# Autodesk Inventor assembly: Noise_ASM
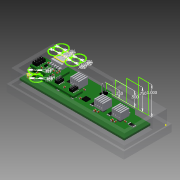
[picture p0: Inventor's stored thumbnail of the model, 180x180]
Saved by Autodesk Inventor 2014 (Build 180170000, 170)
## iProperties
Created: 2015-11-05
Part Number: Noise_ASM
Document SubType Name: Assembly
Designer: Owner
Author: Owner
## Documents named in this file (23)
- C:\Users\Owner\Documents\APC\FrontEnd\IAM\Common\NoiseSource\Noise_ASM.iam
- C:\Users\Owner\Documents\APC\FrontEnd\IAM\Common\NoiseSource\MezzanineBoard.ipt
- C:\Users\Owner\Documents\APC\FrontEnd\IAM\Common\NoiseSource\NoiseBoard.ipt
- C:\Users\Owner\Documents\APC\FrontEnd\IAM\Common\NoiseSource\Header_127.ipt
- C:\Users\Owner\Documents\APC\FrontEnd\IAM\Common\FirstStageAmp.ipt
- C:\Users\Owner\Documents\APC\FrontEnd\IAM\Common\RFSwitch.ipt
- C:\Users\Owner\Documents\APC\FrontEnd\IAM\Common\UMCC.ipt
- C:\Users\Owner\Documents\APC\FrontEnd\IAM\Common\2mm4PosHeader.ipt
- C:\Users\Owner\Documents\APC\FrontEnd\IAM\Common\2mm2Row8PosFemale.ipt
- C:\Users\Owner\Documents\APC\FrontEnd\IAM\Common\Block.ipt
- C:\Users\Owner\Documents\APC\FrontEnd\IAM\Common\2020Resistor.ipt
- C:\Users\Owner\Documents\APC\FrontEnd\IAM\Common\0806Cap.ipt
- C:\Users\Owner\Documents\APC\FrontEnd\IAM\Common\0603Inductor.ipt
- C:\Users\Owner\Documents\APC\FrontEnd\IAM\Common\0603Cap.ipt
- C:\Users\Owner\Documents\APC\FrontEnd\IAM\Common\SmallHeatsink.ipt
- C:\Users\Owner\Documents\APC\FrontEnd\IAM\Common\127mm2Row8PosFemale.ipt
- C:\Users\Owner\Documents\APC\FrontEnd\IAM\Common\2mmWireBoardConn.ipt
- C:\Users\Owner\Documents\APC\FrontEnd\IAM\Common\2mmWireBoardConn_plug.ipt
- C:\Users\Owner\Documents\APC\FrontEnd\IAM\Common\0603Resistor.ipt
- C:\Users\Owner\Documents\APC\FrontEnd\IAM\Common\DualNotGate.ipt
- C:\Users\Owner\Documents\APC\FrontEnd\IAM\Common\UMCC_Plug.ipt
- C:\Users\Owner\Documents\APC\FrontEnd\IAM\Common\2PinHeader.ipt
- C:\Users\Owner\Documents\APC\FrontEnd\IAM\Common\NoiseSourceWell.ipt
## Components (71 placed, 22 different names)
1. MezzanineBoard:1 — Mate:5, Mate:14, Mate:15, Mate:16, Mate:53, Mate:54, Mate:55, Mate:56, Mate:57, Mate:58, Mate:66, Mate:67, Angle:1, Mate:68, Mate:69, Mate:70, Mate:71, Mate:72, Mate:73, Flush:92, Flush:93, Flush:94, Flush:95, Flush:96, Flush:97, Flush:98, Flush:99, Flush:100, Flush:101, Flush:102, Flush:103, Mate:74, Mate:75, Mate:76, Flush:104, Flush:105, Flush:106, Flush:107, Flush:108, Flush:109, Mate:77, Mate:78, Mate:79, Mate:80, Flush:110, Flush:111, Flush:112, Flush:113, Flush:114, Flush:115, Flush:116, Flush:117
2. NoiseBoard:1 — Mate:1, Mate:2, Flush:1, Flush:2, Flush:3, Flush:4, Mate:6, Mate:7, Mate:8, Mate:9, Mate:10, Mate:11, Mate:12, Flush:11, Flush:12, Flush:13, Flush:14, Flush:15, Flush:16, Flush:17, Flush:18, Flush:19, Flush:20, Flush:21, Flush:22, Flush:23, Flush:24, Mate:13, Tangent:1, Tangent:2, Flush:25, Mate:17, Mate:18, Mate:19, Mate:20, Mate:21, Flush:26, Flush:27, Flush:28, Flush:29, Flush:30, Flush:31, Flush:32, Flush:33, Flush:34, Flush:35, Mate:22, Mate:23, Mate:24, Mate:25, Mate:26, Mate:27, Flush:36, Flush:37, Flush:38, Flush:39, Flush:40, Flush:41, Flush:42, Flush:43, Flush:44, Flush:45, Flush:46, Flush:47, Mate:28, Mate:29, Mate:30, Mate:31, Mate:32, Mate:33, Flush:48, Flush:49, Flush:50, Flush:51, Flush:52, Flush:53, Flush:54, Flush:55, Flush:56, Flush:57, Flush:58, Flush:59, Mate:34, Mate:35, Mate:36, Mate:37, Mate:38, Mate:39, Mate:40, Mate:41, Mate:42, Mate:43, Mate:44, Flush:60, Flush:61, Flush:62, Flush:63, Flush:64, Flush:65, Flush:66, Flush:67, Flush:68, Flush:69, Flush:70, Flush:71, Flush:72, Flush:73, Flush:74, Flush:75, Flush:76, Flush:77, Flush:78, Flush:79, Flush:80, Flush:81, Mate:45, Mate:46, Mate:47, Mate:48, Mate:49, Flush:82, Flush:83, Flush:84, Flush:85, Flush:86, Flush:87, Flush:88, Flush:89, Flush:90, Flush:91, Mate:83, Flush:118, Flush:119
3. Header_127:1 — Mate:1, Flush:2, Flush:4, Mate:5, Mate:59, Mate:60
4. Header_127:2 — Mate:2, Flush:1, Flush:3
5. UMCC:1 — Mate:12, Flush:11, Flush:12, Mate:81, Mate:82
6. 2mm4PosHeader:1 — Mate:13, Tangent:1, Tangent:2
7. 2mm2Row8PosFemale:1 — Mate:14, Mate:15, Mate:16
8. Block:1 — Flush:25
9. SmallHeatsink:1 — Mate:50
10. SmallHeatsink:2 — Mate:51
11. SmallHeatsink:3 — Mate:52
12. 127mm2Row8PosFemale:1 — Mate:53, Mate:56, Mate:58
13. 127mm2Row8PosFemale:2 — Mate:54, Mate:55, Mate:57, Mate:59, Mate:60
14. 2mmWireBoardConn:1 — Mate:63, Mate:64, Mate:65, Mate:66, Mate:67, Angle:1
15. 2mmWireBoardConn_plug:1 — Mate:63, Mate:64, Mate:65, Mate:84, Flush:120, Flush:121
16. 0603Resistor:1 — Mate:68, Flush:92, Flush:98
17. 0603Resistor:2 — Mate:69, Flush:93, Flush:100
18. 0603Cap:17 — Mate:70, Flush:95, Flush:99
19. 0603Cap:18 — Mate:71, Flush:96, Flush:101
20. 0603Cap:19 — Mate:73, Flush:97, Flush:103
21. 0603Cap:20 — Mate:72, Flush:94, Flush:102
22. DualNotGate:1 — Mate:75, Flush:105, Flush:107
23. DualNotGate:2 — Mate:76, Flush:104, Flush:109
24. DualNotGate:3 — Mate:74, Flush:106, Flush:108
25. 0603Cap:21 — Mate:77, Flush:116, Flush:117
26. 0603Cap:22 — Mate:78, Flush:114, Flush:115
27. 0603Cap:23 — Mate:79, Flush:112, Flush:113
28. 0603Cap:24 — Mate:80, Flush:110, Flush:111
29. UMCC_Plug:1 — Mate:81, Mate:82
30. 2PinHeader:1 — Mate:83, Flush:118, Flush:119
31. 2mmWireBoardConn_plug:2 — Mate:84, Flush:120, Flush:121
32. NoiseSourceWell:1
33. FirstStageAmp:3 — Mate:8, Flush:22, Flush:24, Mate:52
34. FirstStageAmp:2 — Mate:7, Flush:19, Flush:20, Mate:51
35. FirstStageAmp:1 — Mate:6, Flush:21, Flush:23, Mate:50
36. 2020Resistor:2 — Mate:18, Flush:30, Flush:32
37. 2020Resistor:3 — Mate:19, Flush:34, Flush:35
38. 2020Resistor:4 — Mate:20, Flush:28, Flush:29
39. 0806Cap:1 — Mate:22, Flush:36, Flush:37
40. 0806Cap:2 — Mate:23, Flush:46, Flush:47
41. 0806Cap:3 — Mate:24, Flush:40, Flush:41
42. 0806Cap:4 — Mate:25, Flush:44, Flush:45
43. 0806Cap:5 — Mate:27, Flush:42, Flush:43
44. 0806Cap:6 — Mate:26, Flush:38, Flush:39
45. 0603Inductor:1 — Mate:33, Flush:48, Flush:49
46. 0603Inductor:2 — Mate:32, Flush:50, Flush:51
47. 0603Inductor:3 — Mate:31, Flush:52, Flush:54
48. 0603Inductor:4 — Mate:30, Flush:53, Flush:55
49. 0603Inductor:5 — Mate:29, Flush:56, Flush:58
50. 0603Inductor:6 — Mate:28, Flush:57, Flush:59
51. 0603Cap:1 — Mate:40, Flush:62, Flush:65
52. 0603Cap:2 — Mate:38, Flush:67, Flush:69
53. 0603Cap:3 — Mate:39, Flush:70, Flush:73
54. 0603Cap:4 — Mate:37, Flush:74, Flush:76
55. 0603Cap:5 — Mate:35, Flush:75, Flush:77
56. 0603Cap:6 — Mate:36, Flush:80, Flush:81
57. 0603Cap:7 — Mate:34, Flush:78, Flush:79
58. 0603Cap:8 — Mate:41, Flush:61, Flush:64
59. 0603Cap:9 — Mate:42, Flush:66, Flush:68
60. 0603Cap:10 — Mate:43, Flush:71, Flush:72
61. 0603Cap:11 — Mate:44, Flush:60, Flush:63
62. RFSwitch:2 — Mate:10, Flush:15, Flush:16
63. RFSwitch:1 — Mate:11, Flush:13, Flush:14
64. 0603Cap:12 — Mate:45, Flush:85, Flush:87
65. 0603Cap:15 — Mate:48, Flush:84, Flush:86
66. 0603Cap:13 — Mate:46, Flush:88, Flush:91
67. 0603Cap:14 — Mate:47, Flush:89, Flush:90
68. RFSwitch:3 — Mate:9, Flush:17, Flush:18
69. 2020Resistor:1 — Mate:17, Flush:26, Flush:27
70. 2020Resistor:5 — Mate:21, Flush:31, Flush:33
71. 0603Cap:16 — Mate:49, Flush:82, Flush:83
## Relationships (198: Flush 115, Mate 80, Tangent 2, Angle 1)
- Mate:1: NoiseBoard:1 ↔ Header_127:1
- Mate:2: NoiseBoard:1 ↔ Header_127:2
- Flush:1 (24.5364 mm): NoiseBoard:1 ↔ Header_127:2
- Flush:2 (37.3126 mm): NoiseBoard:1 ↔ Header_127:1
- Flush:3 (6.7564 mm): NoiseBoard:1 ↔ Header_127:2
- Flush:4 (6.8072 mm): NoiseBoard:1 ↔ Header_127:1
- Mate:5: MezzanineBoard:1 ↔ Header_127:1
- Mate:6: NoiseBoard:1 ↔ FirstStageAmp:1
- Mate:7: NoiseBoard:1 ↔ FirstStageAmp:2
- Mate:8: NoiseBoard:1 ↔ FirstStageAmp:3
- Mate:9: NoiseBoard:1 ↔ RFSwitch:3
- Mate:10: NoiseBoard:1 ↔ RFSwitch:2
- Mate:11: NoiseBoard:1 ↔ RFSwitch:1
- Mate:12: NoiseBoard:1 ↔ UMCC:1
- Flush:11 (4.5212 mm): NoiseBoard:1 ↔ UMCC:1
- Flush:12 (2.3368 mm): NoiseBoard:1 ↔ UMCC:1
- Flush:13 (10.5664 mm): NoiseBoard:1 ↔ RFSwitch:1
- Flush:14 (9.0424 mm): NoiseBoard:1 ↔ RFSwitch:1
- Flush:15 (10.5664 mm): NoiseBoard:1 ↔ RFSwitch:2
- Flush:16 (15.1384 mm): NoiseBoard:1 ↔ RFSwitch:2
- Flush:17 (11.0744 mm): NoiseBoard:1 ↔ RFSwitch:3
- Flush:18 (44.6024 mm): NoiseBoard:1 ↔ RFSwitch:3
- Flush:19 (17.1958 mm): NoiseBoard:1 ↔ FirstStageAmp:2
- Flush:20 (33.0962 mm): NoiseBoard:1 ↔ FirstStageAmp:2
- Flush:21 (10.7442 mm): NoiseBoard:1 ↔ FirstStageAmp:1
- Flush:22 (10.7442 mm): NoiseBoard:1 ↔ FirstStageAmp:3
- Flush:23 (61.2648 mm): NoiseBoard:1 ↔ FirstStageAmp:1
- Flush:24 (76.5302 mm): NoiseBoard:1 ↔ FirstStageAmp:3
- Mate:13: NoiseBoard:1 ↔ 2mm4PosHeader:1
- Mate:14: MezzanineBoard:1 ↔ 2mm2Row8PosFemale:1
- Mate:15 (-1.4224 mm): MezzanineBoard:1 ↔ 2mm2Row8PosFemale:1
- Mate:16 (-2.3114 mm): MezzanineBoard:1 ↔ 2mm2Row8PosFemale:1
- Tangent:1 (-12.2134 mm): NoiseBoard:1 ↔ 2mm4PosHeader:1
- Tangent:2 (-1.7232 mm): NoiseBoard:1 ↔ 2mm4PosHeader:1
- Flush:25: NoiseBoard:1 ↔ Block:1
- Mate:17: NoiseBoard:1 ↔ 2020Resistor:1
- Mate:18: NoiseBoard:1 ↔ 2020Resistor:2
- Mate:19: NoiseBoard:1 ↔ 2020Resistor:3
- Mate:20: NoiseBoard:1 ↔ 2020Resistor:4
- Mate:21: NoiseBoard:1 ↔ 2020Resistor:5
- Flush:26 (17.3482 mm): NoiseBoard:1 ↔ 2020Resistor:1
- Flush:27 (9.8044 mm): NoiseBoard:1 ↔ 2020Resistor:1
- Flush:28 (16.8402 mm): NoiseBoard:1 ↔ 2020Resistor:4
- Flush:29 (24.2824 mm): NoiseBoard:1 ↔ 2020Resistor:4
- Flush:30 (52.451 mm): NoiseBoard:1 ↔ 2020Resistor:2
- Flush:31 (84.6582 mm): NoiseBoard:1 ↔ 2020Resistor:5
- Flush:32 (10.3886 mm): NoiseBoard:1 ↔ 2020Resistor:2
- Flush:33 (12.2174 mm): NoiseBoard:1 ↔ 2020Resistor:5
- Flush:34 (10.3632 mm): NoiseBoard:1 ↔ 2020Resistor:3
- Flush:35 (67.7164 mm): NoiseBoard:1 ↔ 2020Resistor:3
- Mate:22: NoiseBoard:1 ↔ 0806Cap:1
- Mate:23: NoiseBoard:1 ↔ 0806Cap:2
- Mate:24: NoiseBoard:1 ↔ 0806Cap:3
- Mate:25: NoiseBoard:1 ↔ 0806Cap:4
- Mate:26: NoiseBoard:1 ↔ 0806Cap:6
- Mate:27: NoiseBoard:1 ↔ 0806Cap:5
- Flush:36 (30.861 mm): NoiseBoard:1 ↔ 0806Cap:1
- Flush:37 (13.208 mm): NoiseBoard:1 ↔ 0806Cap:1
- Flush:38 (29.591 mm): NoiseBoard:1 ↔ 0806Cap:6
- Flush:39 (24.511 mm): NoiseBoard:1 ↔ 0806Cap:6
- Flush:40 (6.5024 mm): NoiseBoard:1 ↔ 0806Cap:3
- Flush:41 (59.055 mm): NoiseBoard:1 ↔ 0806Cap:3
- Flush:42 (20.701 mm): NoiseBoard:1 ↔ 0806Cap:5
- Flush:43 (58.0644 mm): NoiseBoard:1 ↔ 0806Cap:5
- Flush:44 (6.731 mm): NoiseBoard:1 ↔ 0806Cap:4
- Flush:45 (74.295 mm): NoiseBoard:1 ↔ 0806Cap:4
- Flush:46 (20.2946 mm): NoiseBoard:1 ↔ 0806Cap:2
- Flush:47 (75.565 mm): NoiseBoard:1 ↔ 0806Cap:2
- Mate:28: NoiseBoard:1 ↔ 0603Inductor:6
- Mate:29: NoiseBoard:1 ↔ 0603Inductor:5
- Mate:30: NoiseBoard:1 ↔ 0603Inductor:4
- Mate:31: NoiseBoard:1 ↔ 0603Inductor:3
- Mate:32: NoiseBoard:1 ↔ 0603Inductor:2
- Mate:33: NoiseBoard:1 ↔ 0603Inductor:1
- Flush:48 (19.3548 mm): NoiseBoard:1 ↔ 0603Inductor:1
- Flush:49 (31.0388 mm): NoiseBoard:1 ↔ 0603Inductor:1
- Flush:50 (22.5298 mm): NoiseBoard:1 ↔ 0603Inductor:2
- Flush:51 (32.2326 mm): NoiseBoard:1 ↔ 0603Inductor:2
- Flush:52 (12.9032 mm): NoiseBoard:1 ↔ 0603Inductor:3
- Flush:53 (12.9032 mm): NoiseBoard:1 ↔ 0603Inductor:4
- Flush:54 (59.2074 mm): NoiseBoard:1 ↔ 0603Inductor:3
- Flush:55 (74.4728 mm): NoiseBoard:1 ↔ 0603Inductor:4
- Flush:56 (16.0782 mm): NoiseBoard:1 ↔ 0603Inductor:5
- Flush:57 (16.0782 mm): NoiseBoard:1 ↔ 0603Inductor:6
- Flush:58 (60.4012 mm): NoiseBoard:1 ↔ 0603Inductor:5
- Flush:59 (75.6666 mm): NoiseBoard:1 ↔ 0603Inductor:6
- Mate:34: NoiseBoard:1 ↔ 0603Cap:7
- Mate:35: NoiseBoard:1 ↔ 0603Cap:5
- Mate:36: NoiseBoard:1 ↔ 0603Cap:6
- Mate:37: NoiseBoard:1 ↔ 0603Cap:4
- Mate:38: NoiseBoard:1 ↔ 0603Cap:2
- Mate:39: NoiseBoard:1 ↔ 0603Cap:3
- Mate:40: NoiseBoard:1 ↔ 0603Cap:1
- Mate:41: NoiseBoard:1 ↔ 0603Cap:8
- Mate:42: NoiseBoard:1 ↔ 0603Cap:9
- Mate:43: NoiseBoard:1 ↔ 0603Cap:10
- Mate:44: NoiseBoard:1 ↔ 0603Cap:11
- Flush:60 (12.827 mm): NoiseBoard:1 ↔ 0603Cap:11
- Flush:61 (12.827 mm): NoiseBoard:1 ↔ 0603Cap:8
- Flush:62 (12.827 mm): NoiseBoard:1 ↔ 0603Cap:1
- Flush:63 (80.8228 mm): NoiseBoard:1 ↔ 0603Cap:11
- Flush:64 (71.1708 mm): NoiseBoard:1 ↔ 0603Cap:8
- Flush:65 (55.9054 mm): NoiseBoard:1 ↔ 0603Cap:1
- Flush:66 (7.6708 mm): NoiseBoard:1 ↔ 0603Cap:9
- Flush:67 (7.6708 mm): NoiseBoard:1 ↔ 0603Cap:2
- Flush:68 (76.8858 mm): NoiseBoard:1 ↔ 0603Cap:9
- Flush:69 (61.5188 mm): NoiseBoard:1 ↔ 0603Cap:2
- Flush:70 (18.1864 mm): NoiseBoard:1 ↔ 0603Cap:3
- Flush:71 (18.1864 mm): NoiseBoard:1 ↔ 0603Cap:10
- Flush:72 (75.7428 mm): NoiseBoard:1 ↔ 0603Cap:10
- Flush:73 (60.4774 mm): NoiseBoard:1 ↔ 0603Cap:3
- Flush:74 (19.304 mm): NoiseBoard:1 ↔ 0603Cap:4
- Flush:75 (19.304 mm): NoiseBoard:1 ↔ 0603Cap:5
- Flush:76 (37.6428 mm): NoiseBoard:1 ↔ 0603Cap:4
- Flush:77 (27.7368 mm): NoiseBoard:1 ↔ 0603Cap:5
- Flush:78 (14.1478 mm): NoiseBoard:1 ↔ 0603Cap:7
- Flush:79 (33.4518 mm): NoiseBoard:1 ↔ 0603Cap:7
- Flush:80 (24.4348 mm): NoiseBoard:1 ↔ 0603Cap:6
- Flush:81 (32.1818 mm): NoiseBoard:1 ↔ 0603Cap:6
- Mate:45: NoiseBoard:1 ↔ 0603Cap:12
- Mate:46: NoiseBoard:1 ↔ 0603Cap:13
- Mate:47: NoiseBoard:1 ↔ 0603Cap:14
- Mate:48: NoiseBoard:1 ↔ 0603Cap:15
- Mate:49: NoiseBoard:1 ↔ 0603Cap:16
- Flush:82 (4.4958 mm): NoiseBoard:1 ↔ 0603Cap:16
- Flush:83 (6.5786 mm): NoiseBoard:1 ↔ 0603Cap:16
- Flush:84 (10.8966 mm): NoiseBoard:1 ↔ 0603Cap:15
- Flush:85 (10.8966 mm): NoiseBoard:1 ↔ 0603Cap:12
- Flush:86 (3.6576 mm): NoiseBoard:1 ↔ 0603Cap:15
- Flush:87 (5.715 mm): NoiseBoard:1 ↔ 0603Cap:12
- Flush:88 (13.2588 mm): NoiseBoard:1 ↔ 0603Cap:13
- Flush:89 (10.1346 mm): NoiseBoard:1 ↔ 0603Cap:14
- Flush:90 (42.799 mm): NoiseBoard:1 ↔ 0603Cap:14
- Flush:91 (19.9898 mm): NoiseBoard:1 ↔ 0603Cap:13
- Mate:50 (2 mm): SmallHeatsink:1 ↔ FirstStageAmp:1
- Mate:51 (2 mm): SmallHeatsink:2 ↔ FirstStageAmp:2
- Mate:52 (2 mm): SmallHeatsink:3 ↔ FirstStageAmp:3
- Mate:53: MezzanineBoard:1 ↔ 127mm2Row8PosFemale:1
- Mate:54: MezzanineBoard:1 ↔ 127mm2Row8PosFemale:2
- Mate:55 (-2.6924 mm): MezzanineBoard:1 ↔ 127mm2Row8PosFemale:2
- Mate:56 (-2.6416 mm): MezzanineBoard:1 ↔ 127mm2Row8PosFemale:1
- Mate:57 (-3.5814 mm): MezzanineBoard:1 ↔ 127mm2Row8PosFemale:2
- Mate:58 (-16.3576 mm): MezzanineBoard:1 ↔ 127mm2Row8PosFemale:1
- Mate:59 (0.075 mm): Header_127:1 ↔ 127mm2Row8PosFemale:2
- Mate:60 (0.075 mm): Header_127:1 ↔ 127mm2Row8PosFemale:2
- Mate:63: 2mmWireBoardConn:1 ↔ 2mmWireBoardConn_plug:1
- Mate:64: 2mmWireBoardConn:1 ↔ 2mmWireBoardConn_plug:1
- Mate:65: 2mmWireBoardConn:1 ↔ 2mmWireBoardConn_plug:1
- Mate:66: MezzanineBoard:1 ↔ 2mmWireBoardConn:1
- Mate:67: MezzanineBoard:1 ↔ 2mmWireBoardConn:1
- Angle:1 (0 deg): MezzanineBoard:1 ↔ 2mmWireBoardConn:1
- Mate:68: MezzanineBoard:1 ↔ 0603Resistor:1
- Mate:69: MezzanineBoard:1 ↔ 0603Resistor:2
- Mate:70: MezzanineBoard:1 ↔ 0603Cap:17
- Mate:71: MezzanineBoard:1 ↔ 0603Cap:18
- Mate:72: MezzanineBoard:1 ↔ 0603Cap:20
- Mate:73: MezzanineBoard:1 ↔ 0603Cap:19
- Flush:92 (7.239 mm): MezzanineBoard:1 ↔ 0603Resistor:1
- Flush:93 (7.239 mm): MezzanineBoard:1 ↔ 0603Resistor:2
- Flush:94 (7.239 mm): MezzanineBoard:1 ↔ 0603Cap:20
- Flush:95 (5.207 mm): MezzanineBoard:1 ↔ 0603Cap:17
- Flush:96 (5.207 mm): MezzanineBoard:1 ↔ 0603Cap:18
- Flush:97 (5.207 mm): MezzanineBoard:1 ↔ 0603Cap:19
- Flush:98 (11.8618 mm): MezzanineBoard:1 ↔ 0603Resistor:1
- Flush:99 (11.8618 mm): MezzanineBoard:1 ↔ 0603Cap:17
- Flush:100 (14.986 mm): MezzanineBoard:1 ↔ 0603Resistor:2
- Flush:101 (14.986 mm): MezzanineBoard:1 ↔ 0603Cap:18
- Flush:102 (18.034 mm): MezzanineBoard:1 ↔ 0603Cap:20
- Flush:103 (18.034 mm): MezzanineBoard:1 ↔ 0603Cap:19
- Mate:74: MezzanineBoard:1 ↔ DualNotGate:3
- Mate:75: MezzanineBoard:1 ↔ DualNotGate:1
- Mate:76: MezzanineBoard:1 ↔ DualNotGate:2
- Flush:104 (3.9608 mm): MezzanineBoard:1 ↔ DualNotGate:2
- Flush:105 (2.2082 mm): MezzanineBoard:1 ↔ DualNotGate:1
- Flush:106 (5.2562 mm): MezzanineBoard:1 ↔ DualNotGate:3
- Flush:107 (11.5284 mm): MezzanineBoard:1 ↔ DualNotGate:1
- Flush:108 (7.2104 mm): MezzanineBoard:1 ↔ DualNotGate:3
- Flush:109 (2.5876 mm): MezzanineBoard:1 ↔ DualNotGate:2
- Mate:77: MezzanineBoard:1 ↔ 0603Cap:21
- Mate:78: MezzanineBoard:1 ↔ 0603Cap:22
- Mate:79: MezzanineBoard:1 ↔ 0603Cap:23
- Mate:80: MezzanineBoard:1 ↔ 0603Cap:24
- Flush:110 (6.731 mm): MezzanineBoard:1 ↔ 0603Cap:24
- Flush:111 (2.4638 mm): MezzanineBoard:1 ↔ 0603Cap:24
- Flush:112 (7.2898 mm): MezzanineBoard:1 ↔ 0603Cap:23
- Flush:113 (2.159 mm): MezzanineBoard:1 ↔ 0603Cap:23
- Flush:114 (17.7038 mm): MezzanineBoard:1 ↔ 0603Cap:22
- Flush:115 (6.985 mm): MezzanineBoard:1 ↔ 0603Cap:22
- Flush:116 (1.778 mm): MezzanineBoard:1 ↔ 0603Cap:21
- Flush:117 (18.161 mm): MezzanineBoard:1 ↔ 0603Cap:21
- Mate:81: UMCC:1 ↔ UMCC_Plug:1
- Mate:82: UMCC:1 ↔ UMCC_Plug:1
- Mate:83: NoiseBoard:1 ↔ 2PinHeader:1
- Flush:118 (22.0472 mm): NoiseBoard:1 ↔ 2PinHeader:1
- Flush:119 (49.7078 mm): NoiseBoard:1 ↔ 2PinHeader:1
- Mate:84: 2mmWireBoardConn_plug:1 ↔ 2mmWireBoardConn_plug:2
- Flush:120: 2mmWireBoardConn_plug:1 ↔ 2mmWireBoardConn_plug:2
- Flush:121: 2mmWireBoardConn_plug:1 ↔ 2mmWireBoardConn_plug:2
